# Autodesk Inventor assembly: X-belt tensionerShow
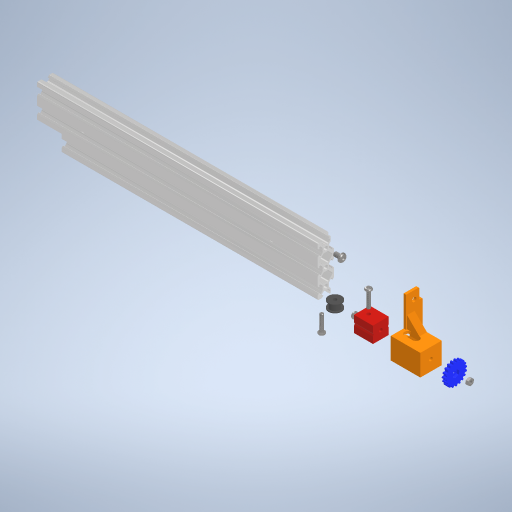
[picture p0: Inventor's stored thumbnail of the model, 512x512]
Saved by Autodesk Inventor 2023 (Build 270158000, 158)
## iProperties
Created: 2023-03-07
Part Number: X-belt tensionerShow
Document SubType Name: Assembly
Designer: Josh
Author: Josh
## Documents named in this file (9)
- C:\Users\Josh\Documents\Inventor\Mingda\X-belt tensionerShow.iam
- C:\Users\Josh\Documents\Inventor\Mingda\X_belt1.ipt
- C:\Users\Josh\Documents\Inventor\Mingda\20x60x342.ipt
- C:\Users\Josh\Documents\Inventor\Mingda\X_belt2.ipt
- C:\Users\Josh\Documents\Inventor\Mingda\Pulley.ipt
- C:\Users\Josh\Documents\Inventor\Content Center Files\R2023\ru-RU\ANSI B18.3.4M(1)\ANSI B18.3.4M - M4 x 0.7 x 20(2).ipt
- C:\Users\Josh\Documents\Inventor\Content Center Files\R2023\ru-RU\ANSI B18.3.4M(1)\ANSI B18.3.4M - M5 x 0.8 x 8(2).ipt
- C:\Users\Josh\Documents\Inventor\Content Center Files\R2023\ru-RU\ANSI B 18.2.4.1 M(1)\ANSI B 18.2.4.1 M - M4 x 0.7Style 1.ipt
- C:\Users\Josh\Documents\Inventor\Mingda\X_belt3.ipt
## Components (10 placed, 8 different names)
1. X_belt1:1 — Совмещение:2, Совмещение:6, Угол:1, Совмещение:14, Угол:3
2. 20x60x342:1 — Совмещение:2, Совмещение:7, Заподлицо:1, Заподлицо:2, Угол:3, Совмещение:15
3. X_belt2:1 — Совмещение:6, Угол:1, Совмещение:13, Совмещение:16, Совмещение:17
4. Pulley:1 — Совмещение:16
5. M4 x 0.7 x 20:1 — Совмещение:13
6. M4 x 0.7 x 20:2 — Совмещение:9, Совмещение:12, Совмещение:17
7. M5 x 0.8 x 8:1 — Совмещение:14
8. M4 x 0.7 x 20:3 — Совмещение:15
9. Hex Nut M4 x 0.7:1 — Угол:2, Совмещение:12
10. X_belt3:1 — Совмещение:9, Угол:2
## Relationships (15: Mate 10, Angle 3, Flush 2)
- Совмещение:2 [Mate]: X_belt1:1 ↔ 20x60x342:1
- Совмещение:6 [Mate]: X_belt1:1 ↔ X_belt2:1
- Совмещение:7 [Mate]: 20x60x342:1
- Заподлицо:1 [Flush]: 20x60x342:1
- Угол:1 [Angle] (0 deg): X_belt1:1 ↔ X_belt2:1
- Заподлицо:2 [Flush]: 20x60x342:1
- Совмещение:9 [Mate]: M4 x 0.7 x 20:2 ↔ X_belt3:1
- Угол:2 [Angle] (0 deg): Hex Nut M4 x 0.7:1 ↔ X_belt3:1
- Совмещение:12 [Mate]: M4 x 0.7 x 20:2 ↔ Hex Nut M4 x 0.7:1
- Совмещение:13 [Mate]: X_belt2:1 ↔ M4 x 0.7 x 20:1
- Совмещение:14 [Mate]: X_belt1:1 ↔ M5 x 0.8 x 8:1
- Совмещение:15 [Mate]: 20x60x342:1 ↔ M4 x 0.7 x 20:3
- Угол:3 [Angle] (0 deg): X_belt1:1 ↔ 20x60x342:1
- Совмещение:16 [Mate]: X_belt2:1 ↔ Pulley:1
- Совмещение:17 [Mate]: X_belt2:1 ↔ M4 x 0.7 x 20:2
